# Autodesk Inventor assembly: woodhouseV1
(part 2 of 2)
- Flush:67: horizontalStrut:2 ↔ horizontalStrut:5
## Named parameters: d17_d10 = 0 mm, d18_d11 = 0 mm, d19_d12 = 0 mm, d20_d13 = 0 mm, d21_d14 = 0 mm, d22_d15 = 0 mm, d23_d16 = 0 mm, d24_d0 = 0 mm, d25_d1 = 0 mm, d26_d2 = 0 mm, d27_d9 = 0 mm, d48_d18 = 0 mm, d49_d19 = 0 mm, d50_d20 = 0 mm, d51_d26 = 0 mm, d57_d17_d10 = 0 mm, d58_d18_d11 = 0 mm, d59_d19_d12 = 0 mm, d60_d20_d13 = 0 mm, d61_d21_d14 = 0 mm, d62_d22_d15 = 0 mm, d63_d23_d16 = 0 mm, d64_d24_d0 = 0 mm, d65_d25_d1 = 0 mm, d66_d26_d2 = 0 mm, d67_d27_d9 = 0 mm, d108_d46 = 0 mm, d109_d48_d18 = 0 mm, d110_d49_d19 = 0 mm, d111_d50_d20 = 0 mm, d112_d51_d26 = 0 mm, d113_d52 = 0 mm, d114_d53 = 0 mm, d115_d54 = 0 mm, d116_d55 = 0 mm, d129_d17_d10 = 0 mm, d130_d18_d11 = 0 mm, d131_d19_d12 = 0 mm, d132_d20_d13 = 0 mm, d133_d21_d14 = 0 mm, d134_d22_d15 = 0 mm, d135_d23_d16 = 0 mm, d136_d24_d0 = 0 mm, d137_d25_d1 = 0 mm, d138_d26_d2 = 0 mm, d139_d27_d9 = 0 mm, d140_d18 = 0 mm, d141_d19 = 0 mm, d142_d20 = 0 mm, d143_d21 = 0 mm, d144_d22 = 0 mm, d145_d23 = 0.5 mm, d147_d26 = 0 mm, d148_d27 = 1 mm, d154_d3 = 0 mm, d155_d4 = 0 mm, d160_d73 = 0 mm, d161_d74 = 0 mm, d162_d0 = 0 mm, d163_d1 = 0 deg, d164_d2 = 102 mm, d169_d73 = 0 mm, d170_d74 = 0 mm, d171_d46 = 0 mm, d172_d48_d18 = 0 mm, d173_d49_d19 = 0 mm, d174_d50_d20 = 0 mm, d175_d51_d26 = 0 mm, d176_d52 = 0 mm, d177_d53 = 0 mm, d178_d54 = 0 mm, d179_d55 = 0 mm, d192_d17_d10 = 0 mm, d193_d18_d11 = 0 mm, d194_d19_d12 = 0 mm, d195_d20_d13 = 0 mm, d196_d21_d14 = 0 mm, d197_d22_d15 = 0 mm, d198_d23_d16 = 0 mm, d199_d24_d0 = 0 mm, d200_d25_d1 = 0 mm, d201_d26_d2 = 0 mm, d202_d27_d9 = 0 mm, d203_d18 = 0 mm, d204_d19 = 0 mm, d205_d20 = 0 mm, d206_d21 = 0 mm, d207_d22 = 0 mm, d208_d23 = 0.5 mm, d209_d24 = 0 mm, d210_d26 = 0 mm, d211_d27 = 1 mm, d212_d28 = 24 mm, d213_d29 = 0 mm, d214_d0 = 0 mm, d215_d1 = 0 deg, d216_d2 = 102 mm, d217_d3 = 0 mm, d218_d4 = 0 mm, d223_d73 = 0 mm, d224_d74 = 0 mm, d225_d46 = 0 mm, d226_d48_d18 = 0 mm, d227_d49_d19 = 0 mm, d228_d50_d20 = 0 mm, d229_d51_d26 = 0 mm, d230_d52 = 0 mm, d231_d53 = 0 mm, d232_d54 = 0 mm, d233_d55 = 0 mm, d246_d17_d10 = 0 mm, d247_d18_d11 = 0 mm, d248_d19_d12 = 0 mm, d249_d20_d13 = 0 mm, d250_d21_d14 = 0 mm, d251_d22_d15 = 0 mm, d252_d23_d16 = 0 mm, d253_d24_d0 = 0 mm, d254_d25_d1 = 0 mm, d255_d26_d2 = 0 mm, d256_d27_d9 = 0 mm, d257_d18 = 0 mm, d258_d19 = 0 mm, d259_d20 = 0 mm, d260_d21 = 0 mm, d261_d22 = 0 mm, d262_d23 = 0.5 mm, d263_d24 = 0 mm, d264_d26 = 0 mm, d265_d27 = 1 mm, d266_d28 = 24 mm, d267_d29 = 0 mm, d268_d0 = 0 mm, d269_d1 = 0 deg, d270_d2 = 102 mm, d271_d3 = 0 mm, d272_d4 = 0 mm, d283_d71 = 0 mm, d320_d276 = 0 mm, d321_d277 = 0 mm, d322_d73 = 0 mm, d323_d74 = 0 mm, d324_d0 = 0 mm, d325_d1 = 0 deg, d326_d2 = 102 mm, d333_d26 = 0 mm, d338_d26 = 0 mm, d343_d72 = 0 mm, d344_d8 = 0 mm, d345_d6 = 0 mm, d346_d41 = 0 deg, d347_d42 = 37 mm, d351_d298 = 0 mm, d352_d299 = 0 mm, d353_d300 = 0 mm, d354_d335 = 0 mm, d355_d336 = 0 mm, d356_d337 = 0 mm, d357_d338_d26 = 0 mm, d358_d339 = 0 mm, d359_d340 = 0 mm, d360_d341 = 0 mm, d361_d342 = 0 mm, d362_d301 = 0 mm, d363_d302 = 0 mm, d364_d303 = 1 mm, d366_d319 = 0 mm, d367_d320_d276 = 0 mm, d368_d321_d277 = 0 mm, d369_d322_d73 = 0 mm, d370_d323_d74 = 0 mm, d371_d324_d0 = 0 mm, d372_d325_d1 = 0 deg, d373_d326_d2 = 102 mm, d374_d327 = 0 mm, d375_d328 = 0 mm, d376_d329 = -2 mm, d377_d330 = 0 mm, d378_d331 = 0 mm, d379_d333_d26 = 0 mm, d380_d334 = 0 mm, d381_d307 = 0 mm, d382_d308 = 0 mm, d383_d309 = 0 mm, d384_d310 = 0 mm, d385_d311 = 0.5 mm, d386_d312 = 0 mm, d387_d313 = 0 mm, d388_d314 = 0 mm, d389_d315 = 0 mm, d390_d316 = 0 mm, d391_d317 = 0 mm, d392_d318 = 0 deg, d393_d298 = 0 mm, d394_d299 = 0 mm, d395_d300 = 0 mm, d396_d335 = 0 mm, d397_d336 = 0 mm, d398_d337 = 0 mm, d399_d338_d26 = 0 mm, d400_d339 = 0 mm, d401_d340 = 0 mm, d402_d341 = 0 mm, d403_d342 = 0 mm, d404_d301 = 0 mm, d405_d302 = 0 mm, d406_d303 = 1 mm, d408_d319 = 0 mm, d409_d320_d276 = 0 mm, d410_d321_d277 = 0 mm, d411_d322_d73 = 0 mm, d412_d323_d74 = 0 mm, d413_d324_d0 = 0 mm, d414_d325_d1 = 0 deg, d415_d326_d2 = 102 mm, d416_d327 = 0 mm, d417_d328 = 0 mm, d418_d329 = -2 mm, d419_d330 = 0 mm, d420_d331 = 0 mm, d421_d333_d26 = 0 mm, d422_d334 = 0 mm, d423_d307 = 0 mm, d424_d308 = 0 mm, d425_d309 = 0 mm, d426_d310 = 0 mm, d427_d311 = 0.5 mm, d428_d312 = 0 mm, d429_d313 = 0 mm, d430_d314 = 0 mm, d431_d315 = 0 mm, d432_d316 = 0 mm, d433_d317 = 0 mm, d434_d318 = 0 deg, d443_d298 = 0 mm, d444_d299 = 0 mm, d445_d300 = 0 mm, d446_d335 = 0 mm, d447_d336 = 0 mm, d448_d337 = 0 mm, d449_d338_d26 = 0 mm, d450_d339 = 0 mm, d451_d340 = 0 mm, d452_d341 = 0 mm, d453_d342 = 0 mm, d454_d301 = 0 mm, d455_d302 = 0 mm, d456_d303 = 1 mm, d458_d319 = 0 mm, d459_d320_d276 = 0 mm, d460_d321_d277 = 0 mm, d461_d322_d73 = 0 mm, d462_d323_d74 = 0 mm, d463_d324_d0 = 0 mm, d464_d325_d1 = 0 deg, d465_d326_d2 = 102 mm, d466_d327 = 0 mm, d467_d328 = 0 mm, d468_d329 = -2 mm, d469_d330 = 0 mm, d470_d331 = 0 mm, d471_d333_d26 = 0 mm, d472_d334 = 0 mm, d473_d307 = 0 mm, d474_d308 = 0 mm, d475_d309 = 0 mm, d476_d310 = 0 mm, d477_d311 = 0.5 mm, d478_d312 = 0 mm, d479_d313 = 0 mm, d480_d314 = 0 mm, d481_d315 = 0 mm, d482_d316 = 0 mm, d483_d317 = 0 mm, d484_d318 = 0 deg, d570_d563 = 0 mm, d571_d564 = 0 mm, d572_d565 = 0 mm, d573_d566 = 0 mm
